# Autodesk Inventor assembly: Assembly2
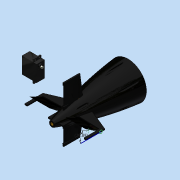
[picture p0: Inventor's stored thumbnail of the model, 180x180]
Saved by Autodesk Inventor 2017 (Build 210142000, 142)
## iProperties
Created: 2016-10-24
Part Number: Assembly2
Document SubType Name: Assembly
Designer: techn
Author: techn
## Documents named in this file (5)
- D:\OneDrive\Documents\Other Projects\Submarine\CAD\aft\Test\MotionTest\Assembly2.iam
- D:\OneDrive\Documents\Other Projects\Submarine\CAD\aft\RearmostAftSectionAssembly0.iam
- D:\OneDrive\Documents\Other Projects\Submarine\CAD\aft\AftSectionWithSteeringLinkages.ipt
- D:\OneDrive\Documents\Other Projects\Submarine\CAD\common\HitecServo\HitecServoAssembly.iam
- D:\OneDrive\Documents\Other Projects\Submarine\CAD\aft\DriveShaft4mm.ipt
## Components (5 placed, 4 different names)
1. RearmostAftSectionAssembly0:1 [sub-assembly] — Mate:1, Mate:2, Angle:2, Mate:3
2. AftSectionWithSteeringLinkages:1 — Mate:1, Mate:2, Angle:1
3. HitecServoAssembly:1 [sub-assembly] — Angle:1, Angle:2
4. HitecServoAssembly:2 [sub-assembly]
5. DriveShaft4mm:1 — Mate:3
## Relationships (5: Mate 3, Angle 2)
- Mate:1: RearmostAftSectionAssembly0:1 ↔ AftSectionWithSteeringLinkages:1
- Mate:2: RearmostAftSectionAssembly0:1 ↔ AftSectionWithSteeringLinkages:1
- Angle:1 (0 deg): AftSectionWithSteeringLinkages:1 ↔ HitecServoAssembly:1
- Angle:2 (0 deg): RearmostAftSectionAssembly0:1 ↔ HitecServoAssembly:1
- Mate:3: RearmostAftSectionAssembly0:1 ↔ DriveShaft4mm:1
